# Autodesk Inventor assembly: TestAssembly
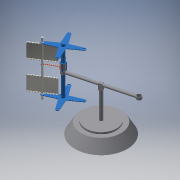
[picture p0: Inventor's stored thumbnail of the model, 180x180]
Saved by Autodesk Inventor 2016 SP1 (Build 200210100, 210)
## iProperties
Created: 2016-02-19
Part Number: TestAssembly
Document SubType Name: Assembly
Designer: Tore Den Store
Author: Tore Den Store
## Documents named in this file (8)
- C:\Users\Jonatan\Documents\Inventor\Vertical axis wind turbine\TestAssembly.iam
- C:\Users\Jonatan\Documents\Inventor\Vertical axis wind turbine\Main\MainBase.ipt
- C:\Users\Jonatan\Documents\Inventor\Vertical axis wind turbine\Main\Centre structure.ipt
- C:\Users\Jonatan\Documents\Inventor\Vertical axis wind turbine\WindPartCentral\WindCentralbeam.ipt
- C:\Users\Jonatan\Documents\Inventor\Vertical axis wind turbine\WindPartRigid 1of2\Rigid holder.ipt
- C:\Users\Jonatan\Documents\Inventor\Vertical axis wind turbine\WindPartCentral\1-of-4-part holder.ipt
- C:\Users\Jonatan\Documents\Inventor\Vertical axis wind turbine\WindPartCentral\Connecting gears.ipt
- C:\Users\Jonatan\Documents\Inventor\Vertical axis wind turbine\1 of 4 part\Assembled.iam
## Components (8 placed, 7 different names)
1. MainBase:1 — Mate:1, Mate:2, Rotational:1
2. Centre structure:1 — Rotational:1, Rigid:1
3. Rigid holder:1 — Rigid:1, Rotational:2, Rotation:1
4. WindCentralbeam:1 — Rotational:2, Cylindrical:1, Mate:4, Mate:7, Rotational:5, Mate:9
5. 1-of-4-part holder:1 — Cylindrical:1, Mate:7, Rotational:6
6. 1-of-4-part holder:2 — Mate:4, Mate:9
7. Connecting gears:1 — Rotational:5, Rotation:1, Rotation:2
8. Assembled:1 [sub-assembly] — Rotational:6, Rotation:2
## Relationships (13: Mate 5, RevoluteJoint 4, RelateRotation 2, WeldJoint 1, CylindricalJoint 1)
- Mate:1: MainBase:1
- Mate:2: MainBase:1
- Rotational:1 [RevoluteJoint]: MainBase:1 ↔ Centre structure:1
- Rigid:1 [WeldJoint]: Centre structure:1 ↔ Rigid holder:1
- Rotational:2 [RevoluteJoint]: Rigid holder:1 ↔ WindCentralbeam:1
- Cylindrical:1: WindCentralbeam:1 ↔ 1-of-4-part holder:1
- Mate:4: WindCentralbeam:1 ↔ 1-of-4-part holder:2
- Mate:7: WindCentralbeam:1 ↔ 1-of-4-part holder:1
- Rotational:5 [RevoluteJoint]: WindCentralbeam:1 ↔ Connecting gears:1
- Rotation:1 [RelateRotation] (1 ul): Rigid holder:1 ↔ Connecting gears:1
- Mate:9: WindCentralbeam:1 ↔ 1-of-4-part holder:2
- Rotational:6 [RevoluteJoint]: 1-of-4-part holder:1 ↔ Assembled:1
- Rotation:2 [RelateRotation] (2 ul): Connecting gears:1 ↔ Assembled:1
